# Autodesk Inventor assembly: one side of drive
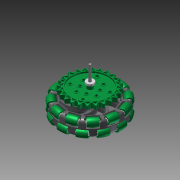
[picture p0: Inventor's stored thumbnail of the model, 180x180]
Saved by Autodesk Inventor 2014 SP1 (Build 180222100, 222)
## iProperties
Created: 2013-08-29
Part Number: one side of drive
Document SubType Name: Assembly
Designer: Ryan
Sending System: SolidWorks 2013
Last Author: Ryan
Author: Ryan
## Documents named in this file (6)
- C:\Users\Ryan\Desktop\sw\toss up 4th robot\drive\wheel assembly.iam
- C:\Users\Ryan\Desktop\sw\lib\Super Sonic Sparks VEX CAD Library\Wheels\4'' Omni-Directional Wheel.iam
- C:\Users\Ryan\Desktop\sw\lib\Aperture VEX CAD Library\Spacers\SPACER-0500-0125.ipt
- C:\Users\Ryan\Desktop\sw\lib\Aperture VEX CAD Library\Hardware\Shaft Collar.ipt
- C:\Users\Ryan\Desktop\sw\lib\Aperture VEX CAD Library\Sprockets\green\High Strength 24-Tooth Sprocket.ipt
- C:\Users\Ryan\Desktop\sw\lib\Aperture VEX CAD Library\Shaft\3 inch Shaft.ipt
## Components (6 placed, 5 different names)
1. LARGE-OMNI-WHEEL:2 [sub-assembly] — Mate:72, Mate:76, Flush:1
2. 2 inch shaft:1 — Mate:81, Mate:82, Flush:1
3. SPACER-0500-0125:1
4. Shaft Collar:1 — Mate:72, Mate:76, Mate:77, Mate:78
5. High Strength 24-Tooth Sprocket:1 — Mate:77, Mate:78, Mate:79, Mate:80, Mate:81, Mate:82
6. SPACER-0500-0125:2 — Mate:79, Mate:80
## Relationships (9: Mate 8, Flush 1)
- Mate:72: LARGE-OMNI-WHEEL:2 ↔ Shaft Collar:1
- Mate:76: LARGE-OMNI-WHEEL:2 ↔ Shaft Collar:1
- Mate:77: Shaft Collar:1 ↔ High Strength 24-Tooth Sprocket:1
- Mate:78: Shaft Collar:1 ↔ High Strength 24-Tooth Sprocket:1
- Mate:79: High Strength 24-Tooth Sprocket:1 ↔ SPACER-0500-0125:2
- Mate:80: High Strength 24-Tooth Sprocket:1 ↔ SPACER-0500-0125:2
- Mate:81: 2 inch shaft:1 ↔ High Strength 24-Tooth Sprocket:1
- Mate:82: 2 inch shaft:1 ↔ High Strength 24-Tooth Sprocket:1
- Flush:1 (-6.35 mm): LARGE-OMNI-WHEEL:2 ↔ 2 inch shaft:1
